# Autodesk Inventor assembly: R2_ハンド
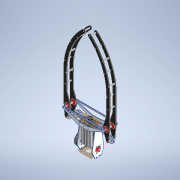
[picture p0: Inventor's stored thumbnail of the model, 180x180]
Saved by Autodesk Inventor 2021 (Build 250183000, 183)
## iProperties
Created: 2021-12-06
Part Number: R2_ハンド
Material: 一般
Document SubType Name: Assembly
Designer: 堀川皓史
Mass: 633.146 g
Surface Area: 2615.18 cm^2
Volume: 339.497 cm^3
Density: 1.86495 g/cm^3
Author: 堀川皓史
## Documents named in this file (14)
- C:\Users\hirohumi\OneDrive\ドキュメント\ロボ研\2022NHKロボコン\R2_version1\R2_ハンド.iam
- C:\Users\hirohumi\OneDrive\ドキュメント\ロボ研\2022NHKロボコン\R2_version1\ハンド_ピストン先.ipt
- C:\Users\hirohumi\OneDrive\ドキュメント\ロボ研\2022NHKロボコン\R2_version1\ハンド_リンク1.ipt
- C:\Users\hirohumi\OneDrive\ドキュメント\ロボ研\2022NHKロボコン\R2_version1\ハンド_上側板.ipt
- C:\Users\hirohumi\OneDrive\ドキュメント\ロボ研\2022NHKロボコン\R2_version1\ハンド.ipt
- C:\Users\hirohumi\OneDrive\ドキュメント\ロボ研\2022NHKロボコン\R2_version1\AIS2017\CDQSB25-40DM(0_1_0).iam
- C:\Users\hirohumi\OneDrive\ドキュメント\ロボ研\2022NHKロボコン\R2_version1\軸_6-24.ipt
- C:\Users\hirohumi\OneDrive\ドキュメント\ロボ研\2022NHKロボコン\R2_version1\軸_6-10.ipt
- C:\Users\hirohumi\OneDrive\ドキュメント\ロボ研\2022NHKロボコン\R2_version1\ベアリング_6-19-6.ipt
- C:\Users\hirohumi\OneDrive\ドキュメント\ロボ研\2022NHKロボコン\R2_version1\3軸アーム\エアシリンダマウント.ipt
- C:\Users\hirohumi\OneDrive\ドキュメント\ロボ研\2022NHKロボコン\R2_version1\3軸アーム\軸6-50.ipt
- C:\Users\hirohumi\OneDrive\ドキュメント\ロボ研\2022NHKロボコン\R2_version1\3軸アーム\エアシリンダ側板.ipt
- C:\Users\hirohumi\OneDrive\ドキュメント\ロボ研\2022NHKロボコン\R2_version1\3軸アーム\プーリ_歯数30.ipt
- C:\Users\hirohumi\OneDrive\ドキュメント\ロボ研\2022NHKロボコン\R2_version1\3軸アーム\ベアリングフランジ付き.ipt
## Components (48 placed, 13 different names)
1. ハンド_ピストン先:1 — メイト:12, メイト:13
2. ハンド_リンク1:1
3. ハンド:1
4. ハンド:2
5. CDQSB25-40DM(0_1_0):1 [sub-assembly] — メイト:12, メイト:13, 挿入:51, 挿入:52
6. 軸_6-24:1
7. 軸_6-10:1
8. 軸_6-10:2
9. ハンド_リンク1:2
10. ハンド_リンク1:3
11. ハンド_リンク1:4
12. ベアリング_6-19-6:1
13. ベアリング_6-19-6:2
14. ベアリング_6-19-6:3
15. ベアリング_6-19-6:4
16. ベアリング_6-19-6:5 — メイト:15
17. ベアリング_6-19-6:6
18. 軸_6-24:2
19. 軸_6-24:3
20. 軸_6-24:4
21. 軸_6-24:5
22. 軸_6-24:6
23. 軸_6-24:7
24. 軸_6-24:8
25. ハンド:3
26. ハンド:4
27. 軸_6-24:9
28. ベアリング_6-19-6:7
29. ベアリング_6-19-6:8 — メイト:14
30. 軸_6-24:10
31. 軸_6-24:11
32. 軸_6-24:12
33. 軸_6-24:13
34. 軸_6-24:14
35. 軸_6-24:15
36. 軸_6-24:16
37. エアシリンダマウント:1 — 挿入:51, 挿入:52, 挿入:53, 挿入:54, 挿入:55, 挿入:56, 挿入:59, 挿入:60, 挿入:61, 挿入:62
38. ハンド_上側板:1 — 挿入:55, 挿入:56
39. ハンド_上側板:2 — 挿入:53, 挿入:54, 挿入:57, 挿入:58
40. 軸6-50:1 — 挿入:57, メイト:15
41. 軸6-50:2 — 挿入:58, メイト:14
42. エアシリンダ側板:1 — 挿入:61, 挿入:62, 挿入:63, 挿入:64, 挿入:67, 挿入:68
43. エアシリンダ側板:2 — 挿入:59, 挿入:60, 挿入:70
44. エアシリンダマウント:2 — 挿入:63, 挿入:64
45. プーリ_歯数30:1 — 挿入:65, 挿入:66, 挿入:67, 挿入:68
46. プーリ_歯数30:2 — 挿入:65, 挿入:66, 挿入:69
47. ベアリングフランジ付き:1 — 挿入:70
48. ベアリングフランジ付き:2 — 挿入:69
## Relationships (66: Insert 54, Mate 12)
- [Insert]: ハンド_ピストン先:1 ↔ 軸_6-10:1
- [Insert]: ハンド_ピストン先:1 ↔ 軸_6-10:2
- [Insert]: ハンド_リンク1:1 ↔ ベアリング_6-19-6:1
- [Insert]: ハンド_リンク1:1 ↔ ベアリング_6-19-6:3
- [Insert]: ハンド_リンク1:2 ↔ ベアリング_6-19-6:2
- [Insert]: ハンド_リンク1:2 ↔ ベアリング_6-19-6:4
- [Insert]: ハンド_リンク1:4 ↔ ベアリング_6-19-6:1
- [Insert]: ハンド_リンク1:4 ↔ ベアリング_6-19-6:3
- [Insert]: ハンド_リンク1:3 ↔ ベアリング_6-19-6:2
- [Insert]: ハンド_リンク1:3 ↔ ベアリング_6-19-6:4
- [Mate]: 軸_6-10:1 ↔ ベアリング_6-19-6:1
- [Mate] (0.5 mm): ハンド_ピストン先:1 ↔ ハンド_リンク1:1
- [Mate]: 軸_6-10:2 ↔ ベアリング_6-19-6:2
- [Mate] (0.5 mm): ハンド_ピストン先:1 ↔ ハンド_リンク1:3
- [Insert]: ハンド:1 ↔ ベアリング_6-19-6:6
- [Insert]: ハンド:2 ↔ ベアリング_6-19-6:5
- [Insert]: ハンド:2 ↔ 軸_6-24:1
- [Insert]: ハンド:2 ↔ 軸_6-24:3
- [Insert]: ハンド:2 ↔ 軸_6-24:5
- [Insert]: ハンド:2 ↔ 軸_6-24:6
- [Insert]: ハンド:2 ↔ 軸_6-24:4
- [Insert]: ハンド:2 ↔ 軸_6-24:2
- [Insert]: ハンド:2 ↔ 軸_6-24:7
- [Insert]: ハンド:1 ↔ 軸_6-24:1
- [Insert]: ハンド:1 ↔ 軸_6-24:3
- [Insert]: ハンド:2 ↔ 軸_6-24:8
- [Insert]: ハンド:3 ↔ ベアリング_6-19-6:8
- [Insert]: ハンド:4 ↔ ベアリング_6-19-6:7
- [Insert]: ハンド:4 ↔ 軸_6-24:9
- [Insert]: ハンド:4 ↔ 軸_6-24:11
- [Insert]: ハンド:4 ↔ 軸_6-24:13
- [Insert]: ハンド:4 ↔ 軸_6-24:14
- [Insert]: ハンド:4 ↔ 軸_6-24:12
- [Insert]: ハンド:4 ↔ 軸_6-24:10
- [Insert]: ハンド:4 ↔ 軸_6-24:15
- [Insert]: ハンド:3 ↔ 軸_6-24:9
- [Insert]: ハンド:3 ↔ 軸_6-24:11
- [Insert]: ハンド:4 ↔ 軸_6-24:16
- [Mate]: ベアリング_6-19-6:4 ↔ 軸_6-24:16
- [Mate] (6 mm): ハンド_リンク1:2 ↔ ハンド:3
- [Mate]: ベアリング_6-19-6:3 ↔ 軸_6-24:8
- [Mate] (6 mm): ハンド:1 ↔ ハンド_リンク1:4
- メイト:12 [Mate]: ハンド_ピストン先:1 ↔ CDQSB25-40DM(0_1_0):1
- メイト:13 [Mate]: ハンド_ピストン先:1 ↔ CDQSB25-40DM(0_1_0):1
- 挿入:51 [Insert]: CDQSB25-40DM(0_1_0):1 ↔ エアシリンダマウント:1
- 挿入:52 [Insert]: CDQSB25-40DM(0_1_0):1 ↔ エアシリンダマウント:1
- 挿入:53 [Insert]: エアシリンダマウント:1 ↔ ハンド_上側板:2
- 挿入:54 [Insert]: エアシリンダマウント:1 ↔ ハンド_上側板:2
- 挿入:55 [Insert]: エアシリンダマウント:1 ↔ ハンド_上側板:1
- 挿入:56 [Insert]: エアシリンダマウント:1 ↔ ハンド_上側板:1
- 挿入:57 [Insert]: ハンド_上側板:2 ↔ 軸6-50:1
- 挿入:58 [Insert]: ハンド_上側板:2 ↔ 軸6-50:2
- メイト:14 [Mate]: ベアリング_6-19-6:8 ↔ 軸6-50:2
- メイト:15 [Mate]: ベアリング_6-19-6:5 ↔ 軸6-50:1
- 挿入:59 [Insert]: エアシリンダマウント:1 ↔ エアシリンダ側板:2
- 挿入:60 [Insert]: エアシリンダマウント:1 ↔ エアシリンダ側板:2
- 挿入:61 [Insert]: エアシリンダマウント:1 ↔ エアシリンダ側板:1
- 挿入:62 [Insert]: エアシリンダマウント:1 ↔ エアシリンダ側板:1
- 挿入:63 [Insert]: エアシリンダ側板:1 ↔ エアシリンダマウント:2
- 挿入:64 [Insert]: エアシリンダ側板:1 ↔ エアシリンダマウント:2
- 挿入:65 [Insert]: プーリ_歯数30:1 ↔ プーリ_歯数30:2
- 挿入:66 [Insert]: プーリ_歯数30:1 ↔ プーリ_歯数30:2
- 挿入:67 [Insert]: エアシリンダ側板:1 ↔ プーリ_歯数30:1
- 挿入:68 [Insert]: エアシリンダ側板:1 ↔ プーリ_歯数30:1
- 挿入:69 [Insert]: プーリ_歯数30:2 ↔ ベアリングフランジ付き:2
- 挿入:70 [Insert]: エアシリンダ側板:2 ↔ ベアリングフランジ付き:1
## Named parameters: d299_d293 = 0 mm, d300_d294 = 0 mm, d301_d295 = 0 mm, d302_d296 = 0 mm, d303_d297 = 0 mm, d304_d298 = 0 mm, d305_d287 = 0 mm, d306_d288 = 0 mm, d307_d289 = 0 mm, d308_d290 = 0 mm, d309_d291 = 0 mm, d310_d292 = 0 mm
